# Autodesk Inventor assembly: guide_bearing_assembly
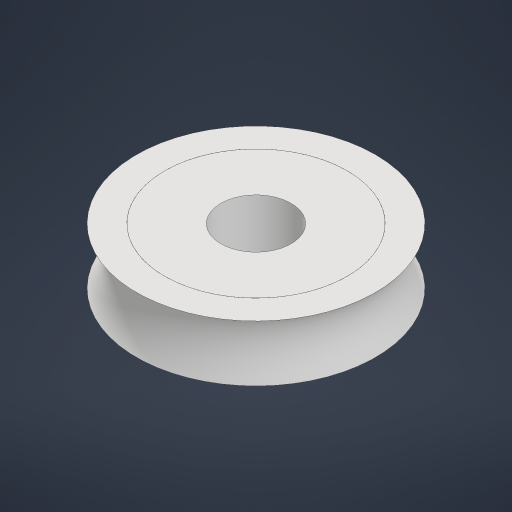
[picture p0: Inventor's stored thumbnail of the model, 512x512]
Saved by Autodesk Inventor 2024 (Build 280153000, 153)
## iProperties
Created: 2026-03-27
Part Number: guide_bearing_assembly
Document SubType Name: Assembly
Designer: schar
Author: schar
## Documents named in this file (3)
- C:\Users\schar\Desktop\FloatingFace\models\guide_bearing_assembly.iam
- C:\Users\schar\Desktop\FloatingFace\models\695_bearing.ipt
- C:\Users\schar\Desktop\FloatingFace\models\guide_profile.ipt
## Components (2 placed, 2 different names)
1. 695_bearing:1 — Mate:1, Flush:1
2. guide_profile:1 — Mate:1, Flush:1
## Relationships (2: Mate 1, Flush 1)
- Mate:1: 695_bearing:1 ↔ guide_profile:1
- Flush:1: 695_bearing:1 ↔ guide_profile:1
